# Autodesk Inventor assembly: A2017_T5_01
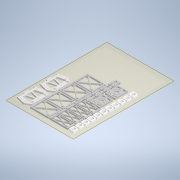
[picture p0: Inventor's stored thumbnail of the model, 180x180]
Saved by Autodesk Inventor 2020 (Build 240168000, 168)
## iProperties
Created: 2021-08-27
Part Number: A2017_T5_01
Document SubType Name: Assembly
Designer: Masato
Author: Masato
## Documents named in this file (8)
- C:\Users\naoki\Documents\Inventor\CitBrains\git_clone\SUSTAINA_ver1_0\OpenPlatform_ver3_0\Cam\A2017_T5_01.iam
- C:\Users\naoki\Documents\Inventor\CitBrains\git_clone\SUSTAINA_ver1_0\OpenPlatform_ver3_0\Cam\DisposableBoard.ipt
- C:\Users\naoki\Documents\Inventor\CitBrains\git_clone\SUSTAINA_ver1_0\OpenPlatform_ver3_0\LowerBody\Knee\Knee_clamp.ipt
- C:\Users\naoki\Documents\Inventor\CitBrains\git_clone\SUSTAINA_ver1_0\OpenPlatform_ver3_0\LowerBody\Foot\Foot_root_block.ipt
- C:\Users\naoki\Documents\Inventor\CitBrains\git_clone\SUSTAINA_ver1_0\OpenPlatform_ver3_0\UpperBody\Trunk\Trunk_lower_side_frame.ipt
- C:\Users\naoki\Documents\Inventor\CitBrains\git_clone\SUSTAINA_ver1_0\OpenPlatform_ver3_0\UpperBody\Arm\Shoulder_horn_frame.ipt
- C:\Users\naoki\Documents\Inventor\CitBrains\git_clone\SUSTAINA_ver1_0\OpenPlatform_ver3_0\LowerBody\Link\FrontLink_diagonal.ipt
- C:\Users\naoki\Documents\Inventor\CitBrains\git_clone\SUSTAINA_ver1_0\OpenPlatform_ver3_0\LowerBody\Link\BackLink_diagonal.ipt
## Components (32 placed, 7 different names)
1. DisposableBoard:1 — メイト:2, メイト:1, フラッシュ:1, フラッシュ:2, メイト:4, メイト:5, メイト:6, メイト:7, メイト:8, メイト:9, フラッシュ:4, フラッシュ:7, 正接:1, 角度:1, フラッシュ:8, 正接:2, メイト:13
2. Shoulder_horn_frame:1 — メイト:8, メイト:18, フラッシュ:9
3. Shoulder_horn_frame:2 — メイト:13, メイト:14, メイト:18, フラッシュ:9, メイト:19
4. FrontLink_diagonal:1 — メイト:6, フラッシュ:4, メイト:10, メイト:12
5. FrontLink_diagonal:2
6. FrontLink_diagonal:3 — メイト:15
7. FrontLink_diagonal:4
8. BackLink_diagonal:1 — メイト:5, メイト:10, フラッシュ:7, 正接:3
9. BackLink_diagonal:2
10. BackLink_diagonal:3
11. BackLink_diagonal:4 — メイト:14, メイト:16
12. Trunk_lower_side_frame:1 — メイト:4, メイト:12, 正接:1, フラッシュ:8
13. Trunk_lower_side_frame:2
14. Foot_root_block:1 — メイト:9, メイト:15, メイト:16
15. Foot_root_block:2
16. Foot_root_block:3
17. Foot_root_block:4
18. Foot_root_block:5
19. Foot_root_block:6 — メイト:19
20. Foot_root_block:7
21. Foot_root_block:8
22. Knee_clamp:1 — メイト:7, 角度:1, 正接:2, 正接:3
23. Knee_clamp:2
24. Knee_clamp:3
25. Knee_clamp:4
26. Knee_clamp:5
27. Knee_clamp:6
28. Knee_clamp:7
29. Knee_clamp:8
30. Knee_clamp:9
31. Knee_clamp:10
32. Knee_clamp:11
## Component patterns: (4 elements, first: FrontLink_diagonal:1), (4 elements, first: BackLink_diagonal:1), (2 elements, first: Trunk_lower_side_frame:1), (8 elements, first: Foot_root_block:1), (11 elements, first: Knee_clamp:1)
## Relationships (26: Mate 16, Flush 6, Tangent 3, Angle 1)
- メイト:2 [Mate]: DisposableBoard:1
- メイト:1 [Mate]: DisposableBoard:1
- フラッシュ:1 [Flush]: DisposableBoard:1
- フラッシュ:2 [Flush]: DisposableBoard:1
- メイト:4 [Mate]: DisposableBoard:1 ↔ Trunk_lower_side_frame:1
- メイト:5 [Mate]: DisposableBoard:1 ↔ BackLink_diagonal:1
- メイト:6 [Mate]: DisposableBoard:1 ↔ FrontLink_diagonal:1
- メイト:7 [Mate]: DisposableBoard:1 ↔ Knee_clamp:1
- メイト:8 [Mate]: DisposableBoard:1 ↔ Shoulder_horn_frame:1
- メイト:9 [Mate]: DisposableBoard:1 ↔ Foot_root_block:1
- フラッシュ:4 [Flush] (2 mm): DisposableBoard:1 ↔ FrontLink_diagonal:1
- メイト:10 [Mate] (2.5 mm): FrontLink_diagonal:1 ↔ BackLink_diagonal:1
- フラッシュ:7 [Flush] (2 mm): DisposableBoard:1 ↔ BackLink_diagonal:1
- メイト:12 [Mate] (2.5 mm): FrontLink_diagonal:1 ↔ Trunk_lower_side_frame:1
- 正接:1 [Tangent] (2 mm): DisposableBoard:1 ↔ Trunk_lower_side_frame:1
- 角度:1 [Angle] (45 deg): DisposableBoard:1 ↔ Knee_clamp:1
- フラッシュ:8 [Flush] (2 mm): DisposableBoard:1 ↔ Trunk_lower_side_frame:1
- 正接:2 [Tangent] (2 mm): DisposableBoard:1 ↔ Knee_clamp:1
- 正接:3 [Tangent] (2.5 mm): BackLink_diagonal:1 ↔ Knee_clamp:1
- メイト:13 [Mate]: DisposableBoard:1 ↔ Shoulder_horn_frame:2
- メイト:14 [Mate] (2.5 mm): Shoulder_horn_frame:2 ↔ BackLink_diagonal:4
- メイト:15 [Mate] (2.5 mm): FrontLink_diagonal:3 ↔ Foot_root_block:1
- メイト:16 [Mate] (2.5 mm): BackLink_diagonal:4 ↔ Foot_root_block:1
- メイト:18 [Mate] (2.5 mm): Shoulder_horn_frame:1 ↔ Shoulder_horn_frame:2
- フラッシュ:9 [Flush]: Shoulder_horn_frame:1 ↔ Shoulder_horn_frame:2
- メイト:19 [Mate] (2.5 mm): Shoulder_horn_frame:2 ↔ Foot_root_block:6
